# Autodesk Inventor assembly: motor_mount1
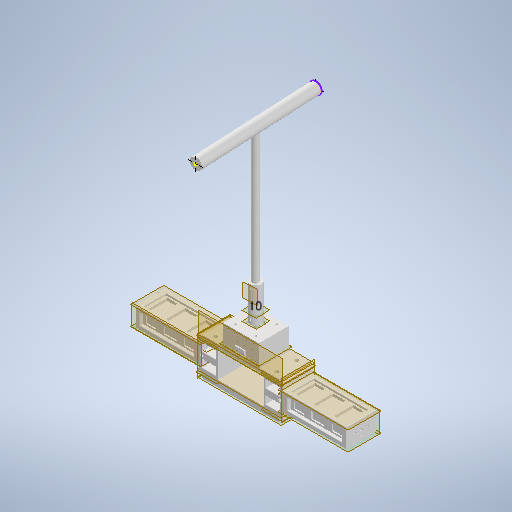
[picture p0: Inventor's stored thumbnail of the model, 512x512]
Saved by Autodesk Inventor 2025.2 (Build 292293000, 293)
## iProperties
Created: 2024-12-30
Part Number: motor_mount1
Document SubType Name: Assembly
Designer: mahhy
Author: mahhy
## Documents named in this file (6)
- D:\兵庫県立大\creap\motor_mount1.iam
- D:\兵庫県立大\creap\motor_rot_born1.ipt
- D:\兵庫県立大\creap\Part7.ipt
- D:\兵庫県立大\creap\motor_mount1.ipt
- D:\兵庫県立大\creap\motor_mount2.ipt
- D:\兵庫県立大\creap\Tonbo.iam
## Components (7 placed, 5 different names)
1. motor_rot_born1:1 — リジッド:1, リジッド:3, リジッド:5
2. motor_rot_born1:2 — リジッド:2, リジッド:4
3. Part7:1 — リジッド:1
4. Part7:2 — リジッド:2
5. motor_mount1:1 — リジッド:3, リジッド:4, リジッド:6
6. motor_mount2:1 — リジッド:5
7. Tonbo:1 [sub-assembly] — リジッド:6
## Relationships (6: WeldJoint 6)
- リジッド:1 [WeldJoint]: motor_rot_born1:1 ↔ Part7:1
- リジッド:2 [WeldJoint]: motor_rot_born1:2 ↔ Part7:2
- リジッド:3 [WeldJoint]: motor_rot_born1:1 ↔ motor_mount1:1
- リジッド:4 [WeldJoint]: motor_rot_born1:2 ↔ motor_mount1:1
- リジッド:5 [WeldJoint]: motor_rot_born1:1 ↔ motor_mount2:1
- リジッド:6 [WeldJoint]: motor_mount1:1 ↔ Tonbo:1
